# Autodesk Inventor assembly: InjectorBoard
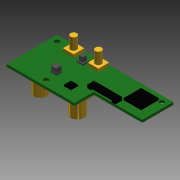
[picture p0: Inventor's stored thumbnail of the model, 180x180]
Saved by Autodesk Inventor 2014 (Build 180170000, 170)
## iProperties
Created: 2015-01-07
Part Number: InjectorBoard
Document SubType Name: Assembly
Designer: Owner
Author: Owner
## Documents named in this file (9)
- C:\Users\Owner\Documents\APC\FrontEnd\IAM\Common\InjectorBoard.iam
- C:\Users\Owner\Documents\APC\FrontEnd\IAM\Common\InjectorBoard.ipt
- C:\Users\Owner\Documents\APC\FrontEnd\IAM\Common\SMA_Up.ipt
- C:\Users\Owner\Documents\APC\FrontEnd\IAM\Common\BNC_Up.ipt
- C:\Users\Owner\Documents\APC\FrontEnd\IAM\Yagi\PIC16Chip.ipt
- C:\Users\Owner\Documents\APC\FrontEnd\IAM\Yagi\FlatFlex26.ipt
- C:\Users\Owner\Documents\APC\FrontEnd\IAM\Yagi\RFSwitch.ipt
- C:\Users\Owner\Documents\APC\FrontEnd\IAM\Yagi\RFCoupler.ipt
- C:\Users\Owner\Documents\APC\FrontEnd\IAM\Yagi\RFSplitter.ipt
## Components (10 placed, 8 different names)
1. InjectorBoard:1 — Mate:1, Mate:2, Mate:3, Mate:4, Mate:5, Mate:6, Mate:7, Flush:1, Flush:2, Flush:3, Flush:4, Flush:5, Flush:6, Flush:7, Flush:8, Flush:9, Flush:10, Flush:11, Flush:12, Flush:13, Flush:14, Flush:15, Flush:16, Flush:17, Flush:18, Flush:19, Flush:20
2. SMA_Up:1 — Mate:1, Flush:6, Flush:9
3. SMA_Up:2 — Mate:2, Flush:7, Flush:8
4. BNC_Up:1 — Mate:6, Flush:2, Flush:4
5. BNC_Up:2 — Mate:7, Flush:1, Flush:3
6. PIC16Chip:1 — Mate:3, Flush:10, Flush:11
7. FlatFlex26:1 — Mate:4, Flush:5, Flush:12
8. RFSwitch:1 — Mate:5, Flush:13, Flush:14
9. RFCoupler:1 — Flush:15, Flush:19, Flush:20
10. RFSplitter:1 — Flush:16, Flush:17, Flush:18
## Relationships (27: Flush 20, Mate 7)
- Mate:1: InjectorBoard:1 ↔ SMA_Up:1
- Mate:2: InjectorBoard:1 ↔ SMA_Up:2
- Mate:3: InjectorBoard:1 ↔ PIC16Chip:1
- Mate:4: InjectorBoard:1 ↔ FlatFlex26:1
- Mate:5: InjectorBoard:1 ↔ RFSwitch:1
- Mate:6: InjectorBoard:1 ↔ BNC_Up:1
- Mate:7: InjectorBoard:1 ↔ BNC_Up:2
- Flush:1 (-3.556 mm): InjectorBoard:1 ↔ BNC_Up:2
- Flush:2 (3.6576 mm): InjectorBoard:1 ↔ BNC_Up:1
- Flush:3 (-1.6256 mm): InjectorBoard:1 ↔ BNC_Up:2
- Flush:4 (-0.889 mm): InjectorBoard:1 ↔ BNC_Up:1
- Flush:5: InjectorBoard:1 ↔ FlatFlex26:1
- Flush:6 (-0.635 mm): InjectorBoard:1 ↔ SMA_Up:1
- Flush:7 (0.635 mm): InjectorBoard:1 ↔ SMA_Up:2
- Flush:8 (11.5062 mm): InjectorBoard:1 ↔ SMA_Up:2
- Flush:9 (27.7622 mm): InjectorBoard:1 ↔ SMA_Up:1
- Flush:10 (3.81 mm): InjectorBoard:1 ↔ PIC16Chip:1
- Flush:11 (5.8928 mm): InjectorBoard:1 ↔ PIC16Chip:1
- Flush:12 (17.6276 mm): InjectorBoard:1 ↔ FlatFlex26:1
- Flush:13 (6.1976 mm): InjectorBoard:1 ↔ RFSwitch:1
- Flush:14 (8.4836 mm): InjectorBoard:1 ↔ RFSwitch:1
- Flush:15: InjectorBoard:1 ↔ RFCoupler:1
- Flush:16: InjectorBoard:1 ↔ RFSplitter:1
- Flush:17 (5.253 mm): InjectorBoard:1 ↔ RFSplitter:1
- Flush:18 (22.017 mm): InjectorBoard:1 ↔ RFSplitter:1
- Flush:19 (19.1516 mm): InjectorBoard:1 ↔ RFCoupler:1
- Flush:20 (9.5504 mm): InjectorBoard:1 ↔ RFCoupler:1
